# Autodesk Inventor assembly: ETL Module Carrier 7pos V1
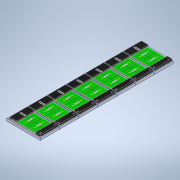
[picture p0: Inventor's stored thumbnail of the model, 180x180]
Saved by Autodesk Inventor 2022 (Build 260153000, 153)
## iProperties
Created: 2022-04-14
Part Number: ETL Module Carrier 7pos V1
Document SubType Name: Assembly
Designer: Caleb
Author: Caleb
## Documents named in this file (7)
- C:\Users\Caleb\Desktop\nebraska-silicon-lab\Hardware\ETL\Module Carrier\Module Carrier V1\ETL Module Carrier 7pos V1.iam
- C:\Users\Caleb\Desktop\nebraska-silicon-lab\Hardware\ETL\modules\tamale v1.3\Tamale - v1p3.iam
- C:\Users\Caleb\Desktop\nebraska-silicon-lab\Hardware\ETL\Module Carrier\Module Carrier V1\Carrier Plate V1.ipt
- C:\Users\Caleb\Desktop\nebraska-silicon-lab\Hardware\ETL\Module Carrier\Module Carrier V1\Carrier Clip V1.ipt
- C:\Users\Caleb\Desktop\nebraska-silicon-lab\Hardware\ETL\Module Carrier\Module Carrier V1\Holder V1.ipt
- C:\Users\Caleb\Desktop\nebraska-silicon-lab\Hardware\ETL\Module Carrier\Module Carrier V1\91771A066_Passivated 18-8 Stainless Steel Phillips Flat Head Screw.ipt
- C:\Users\Caleb\Desktop\nebraska-silicon-lab\Hardware\ETL\Module Carrier\Module Carrier V1\91770A073_Extra-Wide Truss Head Phillips Screws.ipt
## Components (49 placed, 6 different names)
1. Carrier Plate V1:1 — Mate:1, Angle:1, Mate:2, Angle:2, Mate:5, Angle:3, Insert:1, Insert:4
2. Tamale - v1p3:1 [sub-assembly] — Mate:1, Angle:1
3. Holder V1:1 — Mate:5, Angle:3, Insert:1, Insert:2, Insert:3
4. 91771A066_Passivated 18-8 Stainless Steel Phillips Flat Head Screw:1 — Insert:2
5. 91771A066_Passivated 18-8 Stainless Steel Phillips Flat Head Screw:2 — Insert:3
6. Carrier Clip V1:1 — Mate:2, Angle:2
7. 91770A073_Extra-Wide Truss Head Phillips Screws:1 — Insert:4
8. Carrier Plate V1:2
9. Tamale - v1p3:2 [sub-assembly]
10. Holder V1:2
11. 91771A066_Passivated 18-8 Stainless Steel Phillips Flat Head Screw:3
12. 91771A066_Passivated 18-8 Stainless Steel Phillips Flat Head Screw:4
13. Carrier Clip V1:2
14. 91770A073_Extra-Wide Truss Head Phillips Screws:2
15. Carrier Plate V1:3
16. Tamale - v1p3:3 [sub-assembly]
17. Holder V1:3
18. 91771A066_Passivated 18-8 Stainless Steel Phillips Flat Head Screw:5
19. 91771A066_Passivated 18-8 Stainless Steel Phillips Flat Head Screw:6
20. Carrier Clip V1:3
21. 91770A073_Extra-Wide Truss Head Phillips Screws:3
22. Carrier Plate V1:4
23. Tamale - v1p3:4 [sub-assembly]
24. Holder V1:4
25. 91771A066_Passivated 18-8 Stainless Steel Phillips Flat Head Screw:7
26. 91771A066_Passivated 18-8 Stainless Steel Phillips Flat Head Screw:8
27. Carrier Clip V1:4
28. 91770A073_Extra-Wide Truss Head Phillips Screws:4
29. Carrier Plate V1:5
30. Tamale - v1p3:5 [sub-assembly]
31. Holder V1:5
32. 91771A066_Passivated 18-8 Stainless Steel Phillips Flat Head Screw:9
33. 91771A066_Passivated 18-8 Stainless Steel Phillips Flat Head Screw:10
34. Carrier Clip V1:5
35. 91770A073_Extra-Wide Truss Head Phillips Screws:5
36. Carrier Plate V1:6
37. Tamale - v1p3:6 [sub-assembly]
38. Holder V1:6
39. 91771A066_Passivated 18-8 Stainless Steel Phillips Flat Head Screw:11
40. 91771A066_Passivated 18-8 Stainless Steel Phillips Flat Head Screw:12
41. Carrier Clip V1:6
42. 91770A073_Extra-Wide Truss Head Phillips Screws:6
43. Carrier Plate V1:7
44. Tamale - v1p3:7 [sub-assembly]
45. Holder V1:7
46. 91771A066_Passivated 18-8 Stainless Steel Phillips Flat Head Screw:13
47. 91771A066_Passivated 18-8 Stainless Steel Phillips Flat Head Screw:14
48. Carrier Clip V1:7
49. 91770A073_Extra-Wide Truss Head Phillips Screws:7
## Component patterns: (7 elements, first: Carrier Plate V1:1 + Tamale - v1p3:1 + Holder V1:1 + 91771A066_Passivated 18-8 Stainless Steel Phillips Flat Head Screw:1 + 91771A066_Passivated 18-8 Stainless Steel Phillips Flat Head Screw:2 + Carrier Clip V1:1 + 91770A073_Extra-Wide Truss Head Phillips Screws:1)
## Relationships (10: Insert 4, Mate 3, Angle 3)
- Mate:1: Carrier Plate V1:1 ↔ Tamale - v1p3:1
- Angle:1 (0 deg): Carrier Plate V1:1 ↔ Tamale - v1p3:1
- Mate:2: Carrier Plate V1:1 ↔ Carrier Clip V1:1
- Angle:2 (0 deg): Carrier Plate V1:1 ↔ Carrier Clip V1:1
- Mate:5: Carrier Plate V1:1 ↔ Holder V1:1
- Angle:3 (0 deg): Carrier Plate V1:1 ↔ Holder V1:1
- Insert:1: Carrier Plate V1:1 ↔ Holder V1:1
- Insert:2: Holder V1:1 ↔ 91771A066_Passivated 18-8 Stainless Steel Phillips Flat Head Screw:1
- Insert:3: Holder V1:1 ↔ 91771A066_Passivated 18-8 Stainless Steel Phillips Flat Head Screw:2
- Insert:4 (3.5052 mm): Carrier Plate V1:1 ↔ 91770A073_Extra-Wide Truss Head Phillips Screws:1
